# Autodesk Inventor assembly: Сборка8
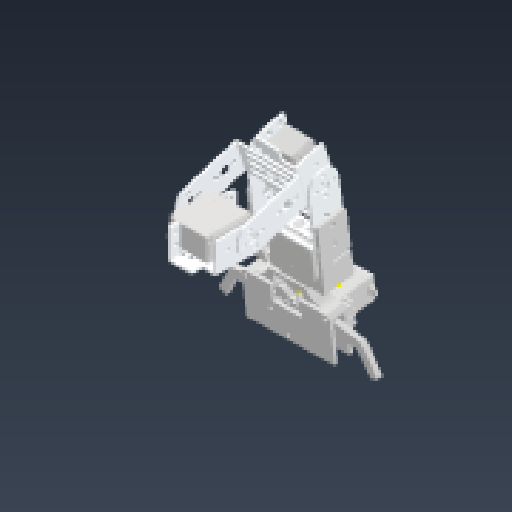
[picture p0: Inventor's stored thumbnail of the model, 512x512]
Saved by Autodesk Inventor 2025 (Build 290162000, 162)
## iProperties
Created: 2025-02-15
Part Number: Сборка8
Document SubType Name: Assembly
Designer: Phantom
Author: Phantom
## Documents named in this file (6)
- C:\Users\GameHD\Desktop\Phantom 16950\Сборка8.iam
- C:\Users\GameHD\Desktop\Phantom 16950\39593_txm-standard-scale pivot armwbearing.ipt
- C:\Users\GameHD\Desktop\Phantom 16950\2000-0025-0002\2000-0025-0002_MIR4_MIR1_MIR.ipt
- C:\Users\GameHD\Desktop\Phantom 16950\для захвата.ipt
- C:\Users\GameHD\Desktop\Phantom 16950\39060_txm-standard servo bracket\39060_txm-standard servo bracket_MIR1.ipt
- C:\Users\GameHD\Desktop\Phantom 16950\захват спереди.iam
## Components (10 placed, 5 different names)
1. 39593_txm-standard-scale pivot armwbearing:1 — Совмещение:1, Совмещение:2, Совмещение:8, Совмещение:17, Совмещение:22, Заподлицо:9, Совмещение:23, Заподлицо:10
2. 2000-0025-0002_MIR4_MIR1_MIR:1 — Совмещение:1, Совмещение:2, Совмещение:16, Совмещение:21, Совмещение:24, Совмещение:25
3. 39060_txm-standard servo bracket_MIR1:2 — Совмещение:8, Совмещение:9, Заподлицо:3, Совмещение:10, Совмещение:12, Заподлицо:5, Заподлицо:6, Совмещение:17
4. 2000-0025-0002_MIR4_MIR1_MIR:2 — Совмещение:9, Заподлицо:3, Совмещение:10
5. 39593_txm-standard-scale pivot armwbearing:2 — Совмещение:12, Заподлицо:5, Заподлицо:6, Совмещение:13, Совмещение:26
6. 39060_txm-standard servo bracket_MIR1:3 — Совмещение:13, Совмещение:15, Заподлицо:8, Совмещение:26
7. 2000-0025-0002_MIR4_MIR1_MIR:3 — Совмещение:15, Заподлицо:8
8. захват спереди:1 [sub-assembly] — Совмещение:16, Совмещение:25
9. для захвата:1 — Совмещение:21, Совмещение:22, Заподлицо:9
10. для захвата:2 — Совмещение:23, Заподлицо:10, Совмещение:24
## Relationships (23: Mate 17, Flush 6)
- Совмещение:1 [Mate]: 39593_txm-standard-scale pivot armwbearing:1 ↔ 2000-0025-0002_MIR4_MIR1_MIR:1
- Совмещение:2 [Mate]: 39593_txm-standard-scale pivot armwbearing:1 ↔ 2000-0025-0002_MIR4_MIR1_MIR:1
- Совмещение:8 [Mate]: 39593_txm-standard-scale pivot armwbearing:1 ↔ 39060_txm-standard servo bracket_MIR1:2
- Совмещение:9 [Mate]: 39060_txm-standard servo bracket_MIR1:2 ↔ 2000-0025-0002_MIR4_MIR1_MIR:2
- Заподлицо:3 [Flush] (1 mm): 39060_txm-standard servo bracket_MIR1:2 ↔ 2000-0025-0002_MIR4_MIR1_MIR:2
- Совмещение:10 [Mate]: 39060_txm-standard servo bracket_MIR1:2 ↔ 2000-0025-0002_MIR4_MIR1_MIR:2
- [Mate]: 39593_txm-standard-scale pivot armwbearing:2 ↔ 39060_txm-standard servo bracket_MIR1:3
- Совмещение:12 [Mate]: 39060_txm-standard servo bracket_MIR1:2 ↔ 39593_txm-standard-scale pivot armwbearing:2
- Заподлицо:5 [Flush] (14 mm): 39060_txm-standard servo bracket_MIR1:2 ↔ 39593_txm-standard-scale pivot armwbearing:2
- Заподлицо:6 [Flush] (-16 mm): 39060_txm-standard servo bracket_MIR1:2 ↔ 39593_txm-standard-scale pivot armwbearing:2
- Совмещение:13 [Mate]: 39593_txm-standard-scale pivot armwbearing:2 ↔ 39060_txm-standard servo bracket_MIR1:3
- Совмещение:15 [Mate]: 39060_txm-standard servo bracket_MIR1:3 ↔ 2000-0025-0002_MIR4_MIR1_MIR:3
- Заподлицо:8 [Flush] (3 mm): 39060_txm-standard servo bracket_MIR1:3 ↔ 2000-0025-0002_MIR4_MIR1_MIR:3
- Совмещение:16 [Mate]: 2000-0025-0002_MIR4_MIR1_MIR:1 ↔ захват спереди:1
- Совмещение:17 [Mate]: 39593_txm-standard-scale pivot armwbearing:1 ↔ 39060_txm-standard servo bracket_MIR1:2
- Совмещение:21 [Mate]: 2000-0025-0002_MIR4_MIR1_MIR:1 ↔ для захвата:1
- Совмещение:22 [Mate]: 39593_txm-standard-scale pivot armwbearing:1 ↔ для захвата:1
- Заподлицо:9 [Flush]: 39593_txm-standard-scale pivot armwbearing:1 ↔ для захвата:1
- Совмещение:23 [Mate]: 39593_txm-standard-scale pivot armwbearing:1 ↔ для захвата:2
- Заподлицо:10 [Flush]: 39593_txm-standard-scale pivot armwbearing:1 ↔ для захвата:2
- Совмещение:24 [Mate]: 2000-0025-0002_MIR4_MIR1_MIR:1 ↔ для захвата:2
- Совмещение:25 [Mate]: 2000-0025-0002_MIR4_MIR1_MIR:1 ↔ захват спереди:1
- Совмещение:26 [Mate]: 39593_txm-standard-scale pivot armwbearing:2 ↔ 39060_txm-standard servo bracket_MIR1:3
## Named parameters: d19_d13 = 0 mm
